# Autodesk Inventor assembly: Link_2
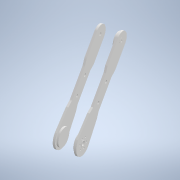
[picture p0: Inventor's stored thumbnail of the model, 180x180]
Saved by Autodesk Inventor 2022 (Build 260153000, 153)
## iProperties
Created: 2021-09-23
Part Number: Link_2
Document SubType Name: Assembly
Designer: Administrador
Author: Administrador
## Documents named in this file (5)
- C:\Users\Administrador\Desktop\Octavo Semestre\Robótica Industrial\Robot\Links\Link_2.iam
- C:\Users\Administrador\Desktop\Octavo Semestre\Robótica Industrial\Robot\Cuerpo\PartesCuerpo\Brazo1.1.ipt
- C:\Users\Administrador\Desktop\Octavo Semestre\Robótica Industrial\Robot\Cuerpo\PartesCuerpo\Estella Servo1.ipt
- C:\Users\Administrador\Desktop\Octavo Semestre\Robótica Industrial\Robot\Cuerpo\PartesCuerpo\Brazo1Izquierda.ipt
- C:\Users\Administrador\Desktop\Octavo Semestre\Robótica Industrial\Robot\Cuerpo\PartesCuerpo\Circulo_Inferior.ipt
## Components (5 placed, 4 different names)
1. Brazo1.1:1
2. Estella Servo1:1
3. Brazo1Izquierda:1
4. Estella Servo1:2
5. Circulo_Inferior:1
## Relationships (8: Mate 8)
- [Mate]: Brazo1.1:1 ↔ Estella Servo1:1
- [Mate]: Brazo1.1:1 ↔ Estella Servo1:1
- [Mate]: Estella Servo1:1 ↔ Brazo1Izquierda:1
- [Mate]: Brazo1.1:1 ↔ Brazo1Izquierda:1
- [Mate]: Brazo1Izquierda:1 ↔ Estella Servo1:2
- [Mate]: Brazo1Izquierda:1 ↔ Estella Servo1:2
- [Mate]: Brazo1Izquierda:1 ↔ Circulo_Inferior:1
- [Mate]: Brazo1Izquierda:1 ↔ Circulo_Inferior:1
